# Autodesk Inventor assembly: 001-FrameBottom
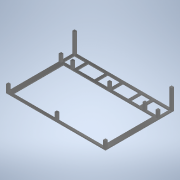
[picture p0: Inventor's stored thumbnail of the model, 180x180]
Saved by Autodesk Inventor 2020 (Build 240168000, 168)
## iProperties
Created: 2019-06-28
Part Number: 001-FrameBottom
Document SubType Name: Assembly
Designer: Mike
Author: Mike
## Documents named in this file (7)
- C:\Users\Mike\Desktop\GitHub\MiZ_LasersaurMod\CAD\001-FrameBottom.iam
- C:\Users\Mike\Desktop\GitHub\MiZ_LasersaurMod\CAD\HFS5-2040-1620.ipt
- C:\Users\Mike\Desktop\GitHub\MiZ_LasersaurMod\CAD\HFS5-2040-1130.ipt
- C:\Users\Mike\Desktop\GitHub\MiZ_LasersaurMod\CAD\HFS5-4040-120.ipt
- C:\Users\Mike\Desktop\GitHub\MiZ_LasersaurMod\CAD\HFS5-2040-860.ipt
- C:\Users\Mike\Desktop\GitHub\MiZ_LasersaurMod\CAD\HFS5-4040-360.ipt
- C:\Users\Mike\Desktop\GitHub\MiZ_LasersaurMod\CAD\HFS5-2040-190.ipt
## Components (22 placed, 6 different names)
1. HFS5-2040-1620:1 — Starr:1, Starr:7, Starr:8, Verschiebbar:4, Verschiebbar:5, Verschiebbar:6, Verschiebbar:7, Starr:15
2. HFS5-2040-1130:1 — Starr:1, Verschiebbar:1, Starr:2, Starr:9
3. HFS5-2040-1130:2 — Starr:3, Starr:10
4. HFS5-2040-1620:2 — Verschiebbar:1, Starr:5, Starr:12, Starr:13, Starr:14, Verschiebbar:2, Verschiebbar:3
5. HFS5-2040-1620:3 — Starr:2, Starr:3, Starr:4, Starr:6, Starr:11
6. HFS5-2040-860:1 — Starr:6
7. HFS5-2040-860:2 — Starr:4, Starr:5
8. HFS5-4040-360:1 — Starr:7
9. HFS5-4040-360:2 — Starr:8
10. HFS5-4040-120:1 — Starr:9
11. HFS5-4040-120:2 — Verschiebbar:3
12. HFS5-4040-120:3 — Verschiebbar:2
13. HFS5-4040-120:4 — Starr:11
14. HFS5-4040-120:5 — Starr:13
15. HFS5-4040-120:6 — Starr:14
16. HFS5-4040-120:7 — Starr:12
17. HFS5-4040-120:8 — Starr:10
18. HFS5-2040-190:1 — Verschiebbar:4
19. HFS5-2040-190:2 — Verschiebbar:5
20. HFS5-2040-190:4 — Verschiebbar:6
21. HFS5-2040-190:5 — Verschiebbar:7
22. HFS5-2040-190:6 — Starr:15
## Relationships (22: WeldJoint 15, TranslationJoint 7)
- Starr:1 [WeldJoint]: HFS5-2040-1620:1 ↔ HFS5-2040-1130:1
- Verschiebbar:1 [TranslationJoint]: HFS5-2040-1130:1 ↔ HFS5-2040-1620:2
- Starr:2 [WeldJoint]: HFS5-2040-1130:1 ↔ HFS5-2040-1620:3
- Starr:3 [WeldJoint]: HFS5-2040-1130:2 ↔ HFS5-2040-1620:3
- Starr:4 [WeldJoint]: HFS5-2040-1620:3 ↔ HFS5-2040-860:2
- Starr:5 [WeldJoint]: HFS5-2040-1620:2 ↔ HFS5-2040-860:2
- Starr:6 [WeldJoint]: HFS5-2040-1620:3 ↔ HFS5-2040-860:1
- Starr:7 [WeldJoint]: HFS5-2040-1620:1 ↔ HFS5-4040-360:1
- Starr:8 [WeldJoint]: HFS5-2040-1620:1 ↔ HFS5-4040-360:2
- Starr:9 [WeldJoint]: HFS5-2040-1130:1 ↔ HFS5-4040-120:1
- Starr:10 [WeldJoint]: HFS5-2040-1130:2 ↔ HFS5-4040-120:8
- Starr:11 [WeldJoint]: HFS5-2040-1620:3 ↔ HFS5-4040-120:4
- Starr:12 [WeldJoint]: HFS5-2040-1620:2 ↔ HFS5-4040-120:7
- Starr:13 [WeldJoint]: HFS5-2040-1620:2 ↔ HFS5-4040-120:5
- Starr:14 [WeldJoint]: HFS5-2040-1620:2 ↔ HFS5-4040-120:6
- Verschiebbar:2 [TranslationJoint]: HFS5-2040-1620:2 ↔ HFS5-4040-120:3
- Verschiebbar:3 [TranslationJoint]: HFS5-2040-1620:2 ↔ HFS5-4040-120:2
- Verschiebbar:4 [TranslationJoint]: HFS5-2040-1620:1 ↔ HFS5-2040-190:1
- Verschiebbar:5 [TranslationJoint]: HFS5-2040-1620:1 ↔ HFS5-2040-190:2
- Verschiebbar:6 [TranslationJoint]: HFS5-2040-1620:1 ↔ HFS5-2040-190:4
- Verschiebbar:7 [TranslationJoint]: HFS5-2040-1620:1 ↔ HFS5-2040-190:5
- Starr:15 [WeldJoint]: HFS5-2040-1620:1 ↔ HFS5-2040-190:6
